# Autodesk Inventor assembly: LilypadV5
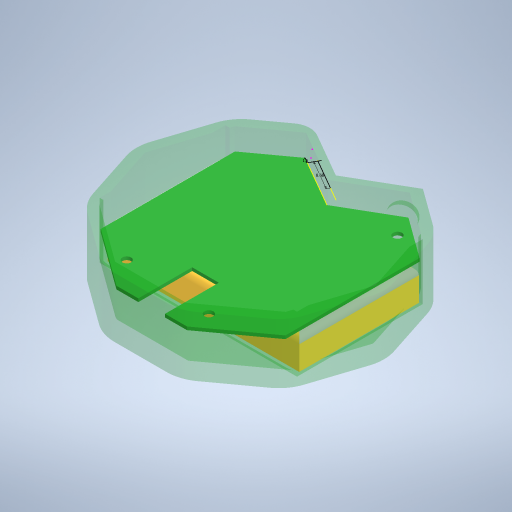
[picture p0: Inventor's stored thumbnail of the model, 512x512]
Saved by Autodesk Inventor 2024 (Build 280153000, 153)
## iProperties
Created: 2023-11-09
Part Number: LilypadV5
Document SubType Name: Assembly
Designer: jevan
Author: jevan
## Documents named in this file (4)
- D:\Windows.old.000\Users\jevan\Documents\Models\Lilypad\V5\LilypadV5.iam
- D:\Windows.old.000\Users\jevan\Documents\Models\Lilypad\V5\ShellMockup_01.ipt
- D:\Windows.old.000\Users\jevan\Documents\Models\Lilypad\V5\Battery.ipt
- D:\Windows.old.000\Users\jevan\Documents\Models\Lilypad\V5\PCB.ipt
## Components (3 placed, 3 different names)
1. ShellMockup_01:1 — Mate:3, Mate:4, Mate:5, Mate:6, Mate:10
2. Battery:1 — Flush:2, Mate:3, Mate:4, Mate:10
3. PCB:1 — Flush:2, Mate:5, Mate:6
## Relationships (6: Mate 5, Flush 1)
- Flush:2: Battery:1 ↔ PCB:1
- Mate:3 (0.75 mm): ShellMockup_01:1 ↔ Battery:1
- Mate:4 (1.3 mm): ShellMockup_01:1 ↔ Battery:1
- Mate:5 (0.25 mm): ShellMockup_01:1 ↔ PCB:1
- Mate:6 (0.25 mm): ShellMockup_01:1 ↔ PCB:1
- Mate:10: ShellMockup_01:1 ↔ Battery:1
